# Autodesk Inventor assembly: UCHWYT PIVOT
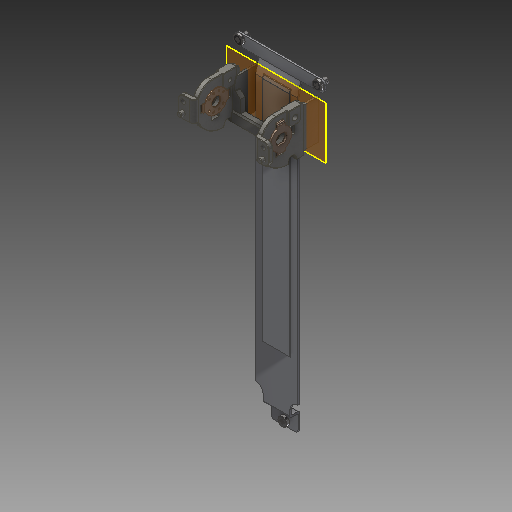
[picture p0: Inventor's stored thumbnail of the model, 512x512]
Saved by Autodesk Inventor 2017 SP1 (Build 210196100, 196)
## iProperties
Created: 2021-02-08
Part Number: UCHWYT PIVOT
Document SubType Name: Assembly
Designer: Napoleon
Author: Napoleon
## Documents named in this file (7)
- D:\PRYWATNE\PROJEKTY\POKÓJ\URZĄDZENIA PERYFERYJNE\DELL 1909Wf\UCHWYT PIVOT.iam
- D:\PRYWATNE\PROJEKTY\POKÓJ\URZĄDZENIA PERYFERYJNE\DELL 1909Wf\UCHWYT KOSZYKA.ipt
- D:\PRYWATNE\PROJEKTY\POKÓJ\URZĄDZENIA PERYFERYJNE\DELL 1909Wf\SŁONECZKO MAŁE.ipt
- D:\PRYWATNE\PROJEKTY\POKÓJ\URZĄDZENIA PERYFERYJNE\DELL 1909Wf\podkładka z jednym uchem.ipt
- D:\PRYWATNE\PROJEKTY\POKÓJ\URZĄDZENIA PERYFERYJNE\DELL 1909Wf\podkładka z dwoma uszami.ipt
- D:\PRYWATNE\PROJEKTY\POKÓJ\URZĄDZENIA PERYFERYJNE\DELL 1909Wf\OSŁONA MECHANIZMU PRZESUWU GÓRA_DÓŁ.ipt
- C:\Users\Administrator\Documents\Inventor\Content Center Files\R2017\pl-pl\Screw GB_T 13806.1-1992 Type A\Screw GB_T 13806.1-1992 A M3 x 4.ipt
## Components (9 placed, 6 different names)
1. UCHWYT KOSZYKA:1 — Zestawiający:1, Zestawiający:2, Zestawiający:3, Równoległy:1, Równoległy:3, Równoległy:4, Zestawiający:9
2. SŁONECZKO MAŁE:1 — Zestawiający:1
3. SŁONECZKO MAŁE:2 — Zestawiający:2
4. podkładka z jednym uchem:1 — Zestawiający:3
5. podkładka z dwoma uszami:1 — Zestawiający:9
6. OSŁONA MECHANIZMU PRZESUWU GÓRA_DÓŁ:1 — Równoległy:2, Równoległy:3, Zestawiający:5, Zestawiający:6, Zestawiający:7, Zestawiający:8, Wstaw:1
7. Screw GB/T 13806.1-1992 Type A M3 x 4:1 — Zestawiający:5, Zestawiający:6
8. Screw GB/T 13806.1-1992 Type A M3 x 4:2 — Zestawiający:7, Zestawiający:8
9. Screw GB/T 13806.1-1992 Type A M3 x 4:3 — Wstaw:1
## Relationships (13: Mate 8, Flush 4, Insert 1)
- Zestawiający:1 [Mate]: UCHWYT KOSZYKA:1 ↔ SŁONECZKO MAŁE:1
- Zestawiający:2 [Mate]: UCHWYT KOSZYKA:1 ↔ SŁONECZKO MAŁE:2
- Zestawiający:3 [Mate]: UCHWYT KOSZYKA:1 ↔ podkładka z jednym uchem:1
- Równoległy:1 [Flush] (-7.5 mm): UCHWYT KOSZYKA:1
- Równoległy:2 [Flush]: OSŁONA MECHANIZMU PRZESUWU GÓRA_DÓŁ:1
- Równoległy:3 [Flush] (-9.5 mm): UCHWYT KOSZYKA:1 ↔ OSŁONA MECHANIZMU PRZESUWU GÓRA_DÓŁ:1
- Równoległy:4 [Flush] (-7.8 mm): UCHWYT KOSZYKA:1
- Zestawiający:5 [Mate]: OSŁONA MECHANIZMU PRZESUWU GÓRA_DÓŁ:1 ↔ Screw GB/T 13806.1-1992 Type A M3 x 4:1
- Zestawiający:6 [Mate]: OSŁONA MECHANIZMU PRZESUWU GÓRA_DÓŁ:1 ↔ Screw GB/T 13806.1-1992 Type A M3 x 4:1
- Zestawiający:7 [Mate]: OSŁONA MECHANIZMU PRZESUWU GÓRA_DÓŁ:1 ↔ Screw GB/T 13806.1-1992 Type A M3 x 4:2
- Zestawiający:8 [Mate]: OSŁONA MECHANIZMU PRZESUWU GÓRA_DÓŁ:1 ↔ Screw GB/T 13806.1-1992 Type A M3 x 4:2
- Wstaw:1 [Insert]: OSŁONA MECHANIZMU PRZESUWU GÓRA_DÓŁ:1 ↔ Screw GB/T 13806.1-1992 Type A M3 x 4:3
- Zestawiający:9 [Mate]: UCHWYT KOSZYKA:1 ↔ podkładka z dwoma uszami:1
